# Autodesk Inventor assembly: terminal assembly
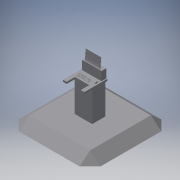
[picture p0: Inventor's stored thumbnail of the model, 180x180]
Saved by Autodesk Inventor 2017 (Build 210142000, 142)
## iProperties
Created: 2018-03-19
Part Number: terminal assembly
Document SubType Name: Assembly
Designer: Braxton
Author: Braxton
## Documents named in this file (5)
- D:\School\Game develpment\geoscape\done\lowend map componts\terminals\assembly\terminal assembly.iam
- D:\School\Game develpment\geoscape\done\lowend map componts\terminals\terminal use.ipt
- D:\School\Game develpment\geoscape\done\lowend map componts\terminals\key board low tec.ipt
- D:\School\Game develpment\geoscape\done\lowend map componts\terminals\terditional mouse.ipt
- D:\School\Game develpment\geoscape\done\lowend map componts\terminals\terminal stand removed rails 2nd map.ipt
## Components (4 placed, 4 different names)
1. terminal use:1 — Mate:14, Mate:15, Mate:16
2. key board low tec:1 — Mate:13, Flush:1, Mate:17, Mate:20
3. terditional mouse:1 — Mate:13, Mate:18, Mate:19
4. terminal stand removed rails 2nd map:1 — Mate:14, Mate:15, Mate:16, Flush:1, Mate:17, Mate:18, Mate:19, Mate:20
## Relationships (9: Mate 8, Flush 1)
- Mate:13: key board low tec:1 ↔ terditional mouse:1
- Mate:14: terminal use:1 ↔ terminal stand removed rails 2nd map:1
- Mate:15: terminal use:1 ↔ terminal stand removed rails 2nd map:1
- Mate:16: terminal use:1 ↔ terminal stand removed rails 2nd map:1
- Flush:1: key board low tec:1 ↔ terminal stand removed rails 2nd map:1
- Mate:17: key board low tec:1 ↔ terminal stand removed rails 2nd map:1
- Mate:18 (-2.1167 mm): terditional mouse:1 ↔ terminal stand removed rails 2nd map:1
- Mate:19: terditional mouse:1 ↔ terminal stand removed rails 2nd map:1
- Mate:20: key board low tec:1 ↔ terminal stand removed rails 2nd map:1
